# Autodesk Inventor assembly: Assembly_Cube_Lens_holder_v3
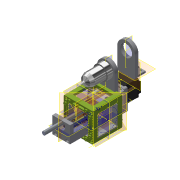
[picture p0: Inventor's stored thumbnail of the model, 180x180]
Saved by Autodesk Inventor 2022 (Build 260153000, 153)
## iProperties
Created: 2020-11-11
Part Number: Assembly_Cube_Lens_holder_v3
Document SubType Name: Assembly
Designer: marsikovabarbora
Author: marsikovabarbora
## Documents named in this file (6)
- C:\Users\PrakashLab\Documents\UC2-Zstage\INVENTOR\Assembly_Cube_Z-Stage_NEMA11_china_v3.iam
- C:\Users\PrakashLab\Documents\UC2-Zstage\INVENTOR\Assembly_Cube_empty_IM_v3.iam
- C:\Users\PrakashLab\Documents\UC2-Zstage\INVENTOR\00_Linear_Stage_NEMA11_china.iam
- C:\Users\PrakashLab\Documents\UC2-Zstage\INVENTOR\00_objectivelens_10x.ipt
- C:\Users\PrakashLab\Documents\UC2-Zstage\INVENTOR\20_Cube_Insert_Cube_Z-Stage_NEMA11_china_objectivemount_v3.ipt
- C:\Users\PrakashLab\Documents\UC2-Zstage\INVENTOR\20_Cube_insert_AlliedVision_Alvium_v3.ipt
## Components (6 placed, 5 different names)
1. 20_Cube_insert_AlliedVision_Alvium_v3:2 — Fluchtend:13, Passend:22
2. 00_objectivelens_10x:1 — Einfügen:3
3. 00_Linear_Stage_NEMA11_china:1 [sub-assembly] — Fluchtend:7, Fluchtend:8, Fluchtend:9, Einfügen:1, Einfügen:2
4. 20_Cube_Insert_Cube_Z-Stage_NEMA11_china_objectivemount_v3:1 — Einfügen:1, Einfügen:2, Einfügen:3
5. Assembly_Cube_empty_IM_v3:2 [sub-assembly] — Fluchtend:7, Fluchtend:8, Fluchtend:9, Fluchtend:13, Passend:22
6. 20_Cube_Insert_Cube_Z-Stage_NEMA11_china_objectivemount_v3:2
## Relationships (8: Flush 4, Insert 3, Mate 1)
- Fluchtend:13 [Flush]: 20_Cube_insert_AlliedVision_Alvium_v3:2 ↔ Assembly_Cube_empty_IM_v3:2
- Passend:22 [Mate]: 20_Cube_insert_AlliedVision_Alvium_v3:2 ↔ Assembly_Cube_empty_IM_v3:2
- Fluchtend:7 [Flush]: 00_Linear_Stage_NEMA11_china:1 ↔ Assembly_Cube_empty_IM_v3:2
- Fluchtend:8 [Flush]: 00_Linear_Stage_NEMA11_china:1 ↔ Assembly_Cube_empty_IM_v3:2
- Fluchtend:9 [Flush] (-47 mm): 00_Linear_Stage_NEMA11_china:1 ↔ Assembly_Cube_empty_IM_v3:2
- Einfügen:1 [Insert]: 00_Linear_Stage_NEMA11_china:1 ↔ 20_Cube_Insert_Cube_Z-Stage_NEMA11_china_objectivemount_v3:1
- Einfügen:2 [Insert]: 00_Linear_Stage_NEMA11_china:1 ↔ 20_Cube_Insert_Cube_Z-Stage_NEMA11_china_objectivemount_v3:1
- Einfügen:3 [Insert]: 00_objectivelens_10x:1 ↔ 20_Cube_Insert_Cube_Z-Stage_NEMA11_china_objectivemount_v3:1
